# Autodesk Inventor assembly: filterWheelAssembly
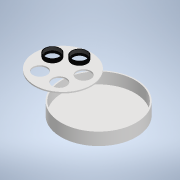
[picture p0: Inventor's stored thumbnail of the model, 180x180]
Saved by Autodesk Inventor 2021 (Build 250183000, 183)
## iProperties
Created: 2020-04-12
Part Number: filterWheelAssembly
Document SubType Name: Assembly
Designer: robst
Author: robst
## Documents named in this file (4)
- C:\git\CAD-Development\robSteele\ShapeWays\TelescopeProjects\FilterWheel\filterWheelAssembly.iam
- C:\git\CAD-Development\robSteele\ShapeWays\TelescopeProjects\FilterWheel\filterBase.ipt
- C:\git\CAD-Development\robSteele\ShapeWays\TelescopeProjects\FilterWheel\filterHolder.ipt
- C:\git\CAD-Development\robSteele\ShapeWays\TelescopeProjects\FilterWheel\simulatedFilter.ipt
## Components (4 placed, 3 different names)
1. filterBase:1
2. filterHolder:1 — Insert:1, Insert:2
3. simulatedFilter:1 — Insert:1
4. simulatedFilter:2 — Insert:2
## Relationships (2: Insert 2)
- Insert:1: filterHolder:1 ↔ simulatedFilter:1
- Insert:2: filterHolder:1 ↔ simulatedFilter:2
